# Autodesk Inventor assembly: AAZLOZENIE
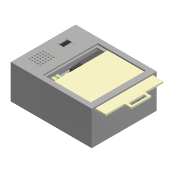
[picture p0: Inventor's stored thumbnail of the model, 180x180]
Saved by Autodesk Inventor 2021 (Build 250183000, 183)
## iProperties
Created: 2022-11-28
Part Number: AAZLOZENIE
Document SubType Name: Assembly
Designer: agnpi
Author: agnpi
## Documents named in this file (22)
- C:\Users\agnpi\Desktop\PLIKI INVENTOR\AAZLOZENIE.iam
- C:\Users\agnpi\Desktop\PLIKI INVENTOR\Podstawa.ipt
- C:\Users\agnpi\Desktop\PLIKI INVENTOR\maly_wentylator.ipt
- C:\Users\agnpi\Desktop\PLIKI INVENTOR\_UCHWYT_DUZY_SILNIK.ipt
- C:\Users\agnpi\Desktop\PLIKI INVENTOR\zlozenie_na_strzykawke_.iam
- C:\Users\agnpi\Desktop\PLIKI INVENTOR\uchwyt_drazki_wersja_2_.ipt
- C:\Users\agnpi\Desktop\PLIKI INVENTOR\uchwyt_maly_silnik_.ipt
- C:\Users\agnpi\Desktop\PLIKI INVENTOR\maly_silnik_.ipt
- C:\Users\agnpi\Desktop\PLIKI INVENTOR\Zlozenie_na_igle_z_nakretka.iam
- C:\Users\agnpi\Desktop\PLIKI INVENTOR\Duzy_silnik_.ipt
- C:\Users\agnpi\Desktop\PLIKI INVENTOR\Zlozenie_prowadnica_na_tlok_nakretka.iam
- C:\Users\agnpi\Desktop\PLIKI INVENTOR\nucleo_746zg_.ipt
- C:\Users\agnpi\Desktop\PLIKI INVENTOR\plytka_stykowa_mala_.ipt
- C:\Users\agnpi\Desktop\PLIKI INVENTOR\krancowka_uchwyt_alternatywa_2_.iam
- C:\Users\agnpi\Desktop\PLIKI INVENTOR\krancowka_.ipt
- C:\Users\agnpi\Desktop\PLIKI INVENTOR\uchwyt_krancowka_alternatywa_2_.ipt
- C:\Users\agnpi\Desktop\PLIKI INVENTOR\Needle.iam
- C:\Users\agnpi\Desktop\PLIKI INVENTOR\Kopula+plus_OLED.iam
- C:\Users\agnpi\Desktop\PLIKI INVENTOR\uchwyt_czujnik.ipt
- C:\Users\agnpi\Desktop\PLIKI INVENTOR\VL6180x_czujnik_.ipt
- C:\Users\agnpi\Desktop\PLIKI INVENTOR\gora_altern_krotsza_z_bolcem.ipt
- C:\Users\agnpi\Desktop\PLIKI INVENTOR\pokrywa_krotsza.ipt
## Components (23 placed, 21 different names)
1. Podstawa:1 — Mate:1, Mate:2, Mate:3, Mate:4, Mate:5, Mate:6, Mate:7, Mate:8, Mate:9, Mate:10, Mate:11, Mate:12, Mate:13, Mate:14, Mate:15, Mate:16, Mate:24, Mate:25, Angle:1, Mate:26, Angle:2, Mate:27, Mate:29, Mate:31, Angle:3, Mate:33, Mate:35, Mate:36, Mate:37, Mate:39, Mate:43, Mate:44, Flush:10, Mate:45
2. maly_wentylator:1 — Mate:1, Mate:2, Mate:3
3. _UCHWYT_DUZY_SILNIK:1 — Mate:4, Mate:5, Mate:6, Mate:20, Mate:21, Mate:22, Mate:28
4. zlozenie_na_strzykawke_:1 [sub-assembly] — Mate:7, Mate:8, Mate:9, Mate:42
5. uchwyt_drazki_wersja_2_:1 — Mate:10, Mate:11, Mate:12, Mate:13
6. uchwyt_maly_silnik_:1 — Mate:14, Mate:15, Mate:16, Mate:17, Mate:18, Mate:19, Mate:32
7. maly_silnik_:1 — Mate:17, Mate:18, Mate:19, Cylindrical:1
8. Zlozenie_na_igle_z_nakretka:1 [sub-assembly] — Cylindrical:1, Flush:2, Flush:5, Mate:34, Flush:6, Mate:40, Mate:41
9. Duzy_silnik_:1 — Mate:20, Mate:21, Mate:22, Cylindrical:2
10. Zlozenie_prowadnica_na_tlok_nakretka:1 [sub-assembly] — Cylindrical:2, Flush:1, Flush:9
11. nucleo_746zg_:1 — Mate:24, Mate:25
12. plytka_stykowa_mala_:1 — Angle:1, Mate:26, Angle:2
13. krancowka_uchwyt_alternatywa_2_:1 [sub-assembly] — Mate:27, Flush:1, Mate:28
14. krancowka_uchwyt_alternatywa_2_:4 [sub-assembly] — Flush:2, Mate:29, Mate:32
15. krancowka_:1 — Flush:3, Flush:4, Mate:30
16. uchwyt_krancowka_alternatywa_2_:1 — Flush:3, Flush:4, Mate:30, Mate:31, Angle:3, Flush:5, Mate:33
17. Needle:1 [sub-assembly] — Mate:34, Flush:6
18. Kopula+plus_OLED:1 [sub-assembly] — Mate:35, Mate:36, Mate:37
19. uchwyt_czujnik:1 — Mate:38, Flush:7, Flush:8, Mate:39
20. VL6180x_czujnik_:1 — Mate:38, Flush:7, Flush:8, Mate:40, Mate:41
21. VL6180x_czujnik_:2 — Mate:42, Flush:9
22. gora_altern_krotsza_z_bolcem:1 — Mate:43, Mate:44, Flush:10, Mate:45, Slider:1
23. pokrywa_krotsza:1 — Slider:1
## Relationships (60: Mate 44, Flush 10, Angle 3, CylindricalJoint 2, TranslationJoint 1)
- Mate:1: Podstawa:1 ↔ maly_wentylator:1
- Mate:2: Podstawa:1 ↔ maly_wentylator:1
- Mate:3: Podstawa:1 ↔ maly_wentylator:1
- Mate:4: Podstawa:1 ↔ _UCHWYT_DUZY_SILNIK:1
- Mate:5: Podstawa:1 ↔ _UCHWYT_DUZY_SILNIK:1
- Mate:6: Podstawa:1 ↔ _UCHWYT_DUZY_SILNIK:1
- Mate:7: Podstawa:1 ↔ zlozenie_na_strzykawke_:1
- Mate:8: Podstawa:1 ↔ zlozenie_na_strzykawke_:1
- Mate:9: Podstawa:1 ↔ zlozenie_na_strzykawke_:1
- Mate:10: Podstawa:1 ↔ uchwyt_drazki_wersja_2_:1
- Mate:11: Podstawa:1 ↔ uchwyt_drazki_wersja_2_:1
- Mate:12: Podstawa:1 ↔ uchwyt_drazki_wersja_2_:1
- Mate:13: Podstawa:1 ↔ uchwyt_drazki_wersja_2_:1
- Mate:14: Podstawa:1 ↔ uchwyt_maly_silnik_:1
- Mate:15: Podstawa:1 ↔ uchwyt_maly_silnik_:1
- Mate:16: Podstawa:1 ↔ uchwyt_maly_silnik_:1
- Mate:17: uchwyt_maly_silnik_:1 ↔ maly_silnik_:1
- Mate:18: uchwyt_maly_silnik_:1 ↔ maly_silnik_:1
- Mate:19: uchwyt_maly_silnik_:1 ↔ maly_silnik_:1
- Cylindrical:1: maly_silnik_:1 ↔ Zlozenie_na_igle_z_nakretka:1
- Mate:20: _UCHWYT_DUZY_SILNIK:1 ↔ Duzy_silnik_:1
- Mate:21: _UCHWYT_DUZY_SILNIK:1 ↔ Duzy_silnik_:1
- Mate:22: _UCHWYT_DUZY_SILNIK:1 ↔ Duzy_silnik_:1
- Cylindrical:2: Duzy_silnik_:1 ↔ Zlozenie_prowadnica_na_tlok_nakretka:1
- Mate:24: Podstawa:1 ↔ nucleo_746zg_:1
- Mate:25 (2 mm): Podstawa:1 ↔ nucleo_746zg_:1
- Angle:1 (90 deg): Podstawa:1 ↔ plytka_stykowa_mala_:1
- Mate:26: Podstawa:1 ↔ plytka_stykowa_mala_:1
- Angle:2 (0 deg): Podstawa:1 ↔ plytka_stykowa_mala_:1
- Mate:27: Podstawa:1 ↔ krancowka_uchwyt_alternatywa_2_:1
- Flush:1: Zlozenie_prowadnica_na_tlok_nakretka:1 ↔ krancowka_uchwyt_alternatywa_2_:1
- Mate:28 (8 mm): _UCHWYT_DUZY_SILNIK:1 ↔ krancowka_uchwyt_alternatywa_2_:1
- Flush:2: Zlozenie_na_igle_z_nakretka:1 ↔ krancowka_uchwyt_alternatywa_2_:4
- Mate:29: Podstawa:1 ↔ krancowka_uchwyt_alternatywa_2_:4
- Flush:3: krancowka_:1 ↔ uchwyt_krancowka_alternatywa_2_:1
- Flush:4: krancowka_:1 ↔ uchwyt_krancowka_alternatywa_2_:1
- Mate:30: krancowka_:1 ↔ uchwyt_krancowka_alternatywa_2_:1
- Mate:31: Podstawa:1 ↔ uchwyt_krancowka_alternatywa_2_:1
- Angle:3 (180 deg): Podstawa:1 ↔ uchwyt_krancowka_alternatywa_2_:1
- Flush:5: Zlozenie_na_igle_z_nakretka:1 ↔ uchwyt_krancowka_alternatywa_2_:1
- Mate:32 (11 mm): uchwyt_maly_silnik_:1 ↔ krancowka_uchwyt_alternatywa_2_:4
- Mate:33 (4 mm): Podstawa:1 ↔ uchwyt_krancowka_alternatywa_2_:1
- Mate:34 (3 mm): Zlozenie_na_igle_z_nakretka:1 ↔ Needle:1
- Flush:6: Zlozenie_na_igle_z_nakretka:1 ↔ Needle:1
- Mate:35: Podstawa:1 ↔ Kopula+plus_OLED:1
- Mate:36: Podstawa:1 ↔ Kopula+plus_OLED:1
- Mate:37: Podstawa:1 ↔ Kopula+plus_OLED:1
- Mate:38: uchwyt_czujnik:1 ↔ VL6180x_czujnik_:1
- Flush:7 (-5 mm): uchwyt_czujnik:1 ↔ VL6180x_czujnik_:1
- Flush:8: uchwyt_czujnik:1 ↔ VL6180x_czujnik_:1
- Mate:39: Podstawa:1 ↔ uchwyt_czujnik:1
- Mate:40 (-1.5 mm): Zlozenie_na_igle_z_nakretka:1 ↔ VL6180x_czujnik_:1
- Mate:41 (2 mm): Zlozenie_na_igle_z_nakretka:1 ↔ VL6180x_czujnik_:1
- Mate:42 (2.5 mm): zlozenie_na_strzykawke_:1 ↔ VL6180x_czujnik_:2
- Flush:9 (8 mm): Zlozenie_prowadnica_na_tlok_nakretka:1 ↔ VL6180x_czujnik_:2
- Mate:43: Podstawa:1 ↔ gora_altern_krotsza_z_bolcem:1
- Mate:44: Podstawa:1 ↔ gora_altern_krotsza_z_bolcem:1
- Flush:10: Podstawa:1 ↔ gora_altern_krotsza_z_bolcem:1
- Mate:45: Podstawa:1 ↔ gora_altern_krotsza_z_bolcem:1
- Slider:1 [TranslationJoint]: gora_altern_krotsza_z_bolcem:1 ↔ pokrywa_krotsza:1
